# Autodesk Inventor assembly: Ontvanger
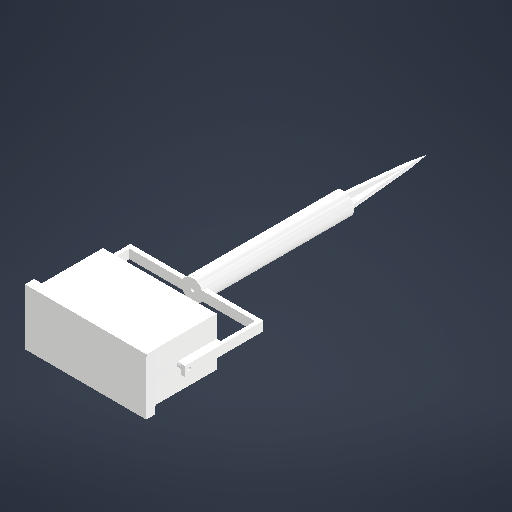
[picture p0: Inventor's stored thumbnail of the model, 512x512]
Saved by Autodesk Inventor 2026.2 (Build 302298000, 298)
## iProperties
Created: 2026-05-05
Part Number: Ontvanger
Document SubType Name: Assembly
Designer: Gameb
Author: Gameb
## Documents named in this file (6)
- C:\Users\Gameb\OneDrive - Stichting Hogeschool Utrecht\Jaar 3\Periode C&D\Quest\11- secor ontwikkeling\3D ontwerp\Zender.iam
- C:\Users\Gameb\OneDrive - Stichting Hogeschool Utrecht\Jaar 3\Periode C&D\Quest\11- secor ontwikkeling\3D ontwerp\Tussen stuk V1.1.ipt
- C:\Users\Gameb\OneDrive - Stichting Hogeschool Utrecht\Jaar 3\Periode C&D\Quest\11- secor ontwikkeling\3D ontwerp\Prikker V1.1.ipt
- C:\Users\Gameb\OneDrive - Stichting Hogeschool Utrecht\Jaar 3\Periode C&D\Quest\11- secor ontwikkeling\3D ontwerp\Sensor houder.ipt
- C:\Users\Gameb\OneDrive - Stichting Hogeschool Utrecht\Jaar 3\Periode C&D\Quest\11- secor ontwikkeling\3D ontwerp\Bakje laser.ipt
- C:\Users\Gameb\OneDrive - Stichting Hogeschool Utrecht\Jaar 3\Periode C&D\Quest\11- secor ontwikkeling\3D ontwerp\Deksel laser.ipt
## Components (5 placed, 5 different names)
1. Prikker V1.1:1 — Mate:4
2. Sensor houder:1 — Mate:3, Mate:7
3. Tussen stuk V1.1:1 — Mate:3, Mate:4
4. Bakje laser:1 — Mate:5, Mate:6, Mate:7, Mate:8
5. Deksel laser:1 — Mate:5, Mate:6, Mate:8
## Relationships (6: Mate 6)
- Mate:3: Sensor houder:1 ↔ Tussen stuk V1.1:1
- Mate:4: Prikker V1.1:1 ↔ Tussen stuk V1.1:1
- Mate:5: Bakje laser:1 ↔ Deksel laser:1
- Mate:6: Bakje laser:1 ↔ Deksel laser:1
- Mate:7: Sensor houder:1 ↔ Bakje laser:1
- Mate:8: Bakje laser:1 ↔ Deksel laser:1
